# Autodesk Inventor assembly: SonyQX_Mechanik
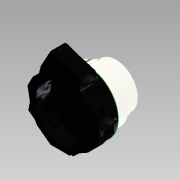
[picture p0: Inventor's stored thumbnail of the model, 180x180]
Saved by Autodesk Inventor 2015 (Build 190159000, 159)
## iProperties
Created: 2015-10-11
Part Number: SonyQX_Mechanik
Document SubType Name: Assembly
Designer: Bene
Author: Bene
## Documents named in this file (3)
- C:\Users\Bene\Dropbox\Dokumente\FHKoeln\Projekt_OE\Inventor\HoloscopeRaspberry\SonyQX_Mechanik.iam
- C:\Users\Bene\Dropbox\Dokumente\FHKoeln\Projekt_OE\Inventor\HoloscopeRaspberry\01_Objektiv.ipt
- C:\Users\Bene\Dropbox\Dokumente\FHKoeln\Projekt_OE\Inventor\HoloscopeRaspberry\02_Ring_1.ipt
## Components (2 placed, 2 different names)
1. 01_Objektiv:1
2. 02_Ring_1:1
## Relationships (1: Flush 1)
- [Flush]: 01_Objektiv:1 ↔ 02_Ring_1:1
